# Autodesk Inventor assembly: VF65-ICF114-adapter
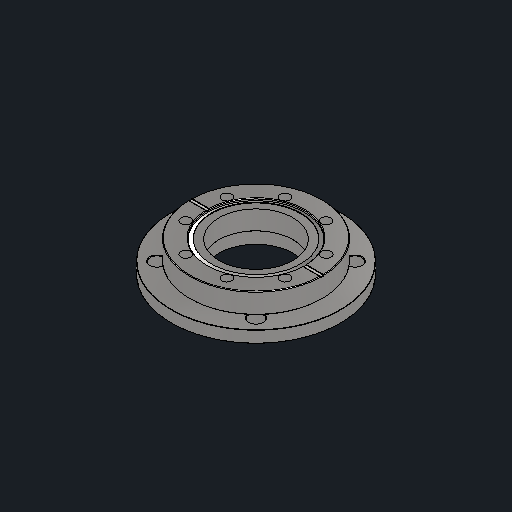
[picture p0: Inventor's stored thumbnail of the model, 512x512]
Saved by Autodesk Inventor 2026 (Build 300175050, 175E)
## iProperties
Created: 2026-01-06
Part Number: VF65-ICF114-adapter
Document SubType Name: Assembly
Designer: queezz
Author: queezz
## Documents named in this file (3)
- C:\Users\queezz\Dropbox\Drawings\PIHTI\TMP-PT-50\VF65-ICF114-adapter.iam
- C:\Users\queezz\Dropbox\Drawings\PIHTI\ContentCenter\CF-parts\CF-Flanges\cf114_blank.ipt
- C:\Users\queezz\Dropbox\Drawings\PIHTI\ContentCenter\JIS-flanges\JIS-VG65.ipt
## Components (2 placed, 2 different names)
1. cf114_blank:1 — Mate:1, Mate:2, Flush:1, Flush:2, Mate:3
2. JIS-VG65:1 — Mate:1, Mate:2, Angle:1
## Relationships (6: Mate 3, Flush 2, Angle 1)
- Mate:1: cf114_blank:1 ↔ JIS-VG65:1
- Mate:2: cf114_blank:1 ↔ JIS-VG65:1
- Flush:1: cf114_blank:1
- Flush:2: cf114_blank:1
- Mate:3: cf114_blank:1
- Angle:1 (45 deg): JIS-VG65:1
